# Autodesk Inventor assembly: Castor
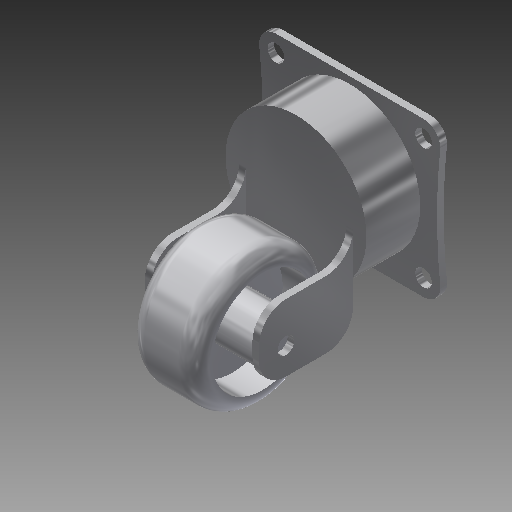
[picture p0: Inventor's stored thumbnail of the model, 512x512]
Saved by Autodesk Inventor 2018 (Build 220112000, 112)
## iProperties
Created: 2018-01-12
Part Number: Castor
Document SubType Name: Assembly
Designer: Kyle
Author: Kyle
## Documents named in this file (3)
- C:\Users\Kyle-HP\Documents\Hackathon-2018\Inventor\Robot\Castor.iam
- C:\Users\Kyle-HP\Documents\Hackathon-2018\Inventor\Robot\CastorBase.ipt
- C:\Users\Kyle-HP\Documents\Hackathon-2018\Inventor\Robot\CastorWheel.ipt
## Components (2 placed, 2 different names)
1. CastorBase:1 — Mate:1, Mate:2
2. CastorWheel:1 — Mate:1, Mate:2
## Relationships (2: Mate 2)
- Mate:1: CastorBase:1 ↔ CastorWheel:1
- Mate:2: CastorBase:1 ↔ CastorWheel:1
